# Autodesk Inventor assembly: ASY PNS 1000 MAIN FRAME
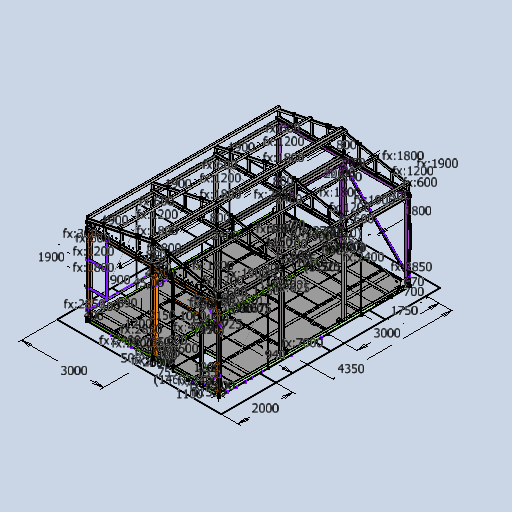
[picture p0: Inventor's stored thumbnail of the model, 512x512]
Saved by Autodesk Inventor 2025 (Build 290162010, 162A)
## iProperties
Created: 2025-03-10
Part Number: ASY PNS 1000 MAIN FRAME
Document SubType Name: Assembly
Designer: admin
Mass: 2.8663e+06 g
Surface Area: 2.46536e+06 cm^2
Volume: 364070 cm^3
Density: 7.87293 g/cm^3
Author: admin
## Documents named in this file (6)
- C:\Users\user\YandexDisk-badmisterfox\home pc\Inventor\PNS2-Panaevsk\ASY PNS 1000 MAIN FRAME.iam
- C:\Users\user\YandexDisk-badmisterfox\home pc\Inventor\PNS2-Panaevsk\PNS-1100 FRAME Main sketch.ipt
- C:\Users\user\YandexDisk-badmisterfox\home pc\Inventor\PNS2-Panaevsk\ASY PNS 1300 frame roof.iam
- C:\Users\user\YandexDisk-badmisterfox\home pc\Inventor\PNS2-Panaevsk\ASY PNS 1100 left module.iam
- C:\Users\user\YandexDisk-badmisterfox\home pc\Inventor\PNS2-Panaevsk\ASY PNS 1200 right module.iam
- C:\Users\user\YandexDisk-badmisterfox\home pc\Inventor\PNS2-Panaevsk\PNS-0265 roof beam.ipt
## Components (13 placed, 5 different names)
1. PNS-0100 FRAME Main sketch:1
2. ASY PNS-0170 frame roof:1 [sub-assembly] — Flush:11, Mate:5, Flush:12
3. ASY PNS-0170 frame roof:2 [sub-assembly]
4. ASY PNS-0170 frame roof:3 [sub-assembly]
5. ASY PNS-0170 frame roof:4 [sub-assembly] — Rigid:14, Rigid:15, Rigid:16, Rigid:17, Rigid:18
6. ASY PNS-001 left module:1 [sub-assembly] — Flush:12
7. ASY PNS-002 right module:1 [sub-assembly] — Mate:5
8. PNS-0265 roof beam:1
9. PNS-0265 roof beam:2 — Rigid:14
10. PNS-0265 roof beam:3 — Rigid:15
11. PNS-0265 roof beam:4 — Rigid:16
12. PNS-0265 roof beam:5 — Rigid:17
13. PNS-0265 roof beam:6 — Rigid:18
## Relationships (21: WeldJoint 9, Flush 8, Mate 4)
- [Flush]: ASY PNS-001 left module:1
- [Flush]: ASY PNS-001 left module:1
- [Flush]: ASY PNS-001 left module:1
- [WeldJoint]: ASY PNS-001 left module:1 ↔ ASY PNS-002 right module:1
- [WeldJoint]: ASY PNS-001 left module:1 ↔ ASY PNS-002 right module:1
- [Mate]: ASY PNS-0170 frame roof:2 ↔ ASY PNS-002 right module:1
- [Mate]: ASY PNS-0170 frame roof:3 ↔ ASY PNS-002 right module:1
- [Mate]: ASY PNS-0170 frame roof:4 ↔ ASY PNS-002 right module:1
- [Flush]: ASY PNS-0170 frame roof:4 ↔ ASY PNS-002 right module:1
- [Flush]: ASY PNS-0170 frame roof:3 ↔ ASY PNS-002 right module:1
- [Flush]: ASY PNS-0170 frame roof:2 ↔ ASY PNS-002 right module:1
- [WeldJoint]: ASY PNS-001 left module:1 ↔ ASY PNS-002 right module:1
- [WeldJoint]: ASY PNS-0170 frame roof:1 ↔ PNS-0265 roof beam:1
- Rigid:14 [WeldJoint]: ASY PNS-0170 frame roof:4 ↔ PNS-0265 roof beam:2
- Rigid:15 [WeldJoint]: ASY PNS-0170 frame roof:4 ↔ PNS-0265 roof beam:3
- Rigid:16 [WeldJoint]: ASY PNS-0170 frame roof:4 ↔ PNS-0265 roof beam:4
- Rigid:17 [WeldJoint]: ASY PNS-0170 frame roof:4 ↔ PNS-0265 roof beam:5
- Rigid:18 [WeldJoint]: ASY PNS-0170 frame roof:4 ↔ PNS-0265 roof beam:6
- Flush:11: ASY PNS-0170 frame roof:1
- Mate:5: ASY PNS-0170 frame roof:1 ↔ ASY PNS-002 right module:1
- Flush:12: ASY PNS-0170 frame roof:1 ↔ ASY PNS-001 left module:1
